# Autodesk Inventor assembly: Motor and Bracket_MIR
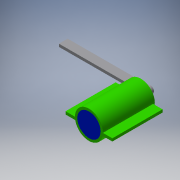
[picture p0: Inventor's stored thumbnail of the model, 180x180]
Saved by Autodesk Inventor 2016 SP1 (Build 200210100, 210)
## iProperties
Created: 2016-04-13
Part Number: Motor and Bracket_MIR
Document SubType Name: Assembly
Designer: schiu30
Author: schiu30
## Documents named in this file (4)
- \\prism.nas.gatech.edu\schiu30\vlab\desktop\Capstone\Capstone CAD\Capstone CAD\Motor + Attachment\Motor and Bracket_MIR.iam
- \\prism.nas.gatech.edu\schiu30\vlab\desktop\Capstone\Capstone CAD\Capstone CAD\Motor + Attachment\Attachment2_MIR.ipt
- \\prism.nas.gatech.edu\schiu30\vlab\desktop\Capstone\Capstone CAD\Capstone CAD\Motor + Attachment\Rotator2_MIR.ipt
- \\prism.nas.gatech.edu\schiu30\vlab\desktop\Capstone\Capstone CAD\Capstone CAD\Motor + Attachment\Motor + Shaft_MIR.iam
## Components (3 placed, 3 different names)
1. Attachment2_MIR:1 — Flush:3, Flush:2, Flush:1, Insert:1
2. Rotator2_MIR:1 — Mate:1, Flush:4
3. Motor + Shaft_MIR:1 [sub-assembly] — Mate:1, Flush:4, Insert:1
## Relationships (6: Flush 4, Mate 1, Insert 1)
- Flush:3: Attachment2_MIR:1
- Flush:2: Attachment2_MIR:1
- Flush:1: Attachment2_MIR:1
- Mate:1: Rotator2_MIR:1 ↔ Motor + Shaft_MIR:1
- Flush:4 (-1.016 mm): Rotator2_MIR:1 ↔ Motor + Shaft_MIR:1
- Insert:1: Attachment2_MIR:1 ↔ Motor + Shaft_MIR:1
